# Autodesk Inventor assembly: Zebro_lotka
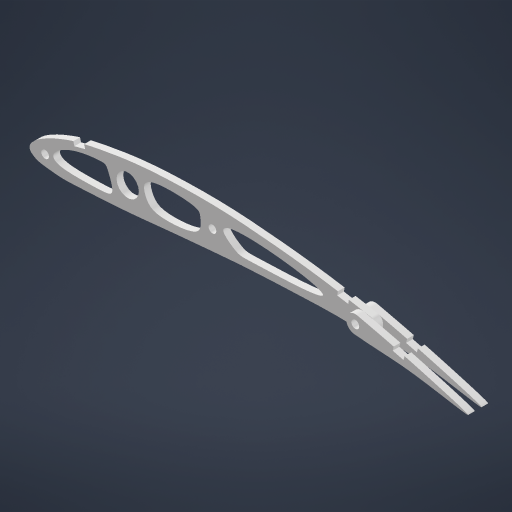
[picture p0: Inventor's stored thumbnail of the model, 512x512]
Saved by Autodesk Inventor 2023 (Build 270158000, 158)
## iProperties
Created: 2023-01-05
Part Number: Zebro_lotka
Document SubType Name: Assembly
Designer: szykr
Author: szykr
## Documents named in this file (3)
- D:\Folder Instalacyjny\GitHub Pliki\Solaris\new model\Zebro_lotka.iam
- D:\Folder Instalacyjny\GitHub Pliki\Solaris\new model\Żebro z lotką.ipt
- D:\Folder Instalacyjny\GitHub Pliki\Solaris\new model\Lotka.ipt
## Components (3 placed, 2 different names)
1. Żebro z lotką:1 — Rotational:1, Rotational:2
2. Lotka:1 — Rotational:2, Angle:1
3. Lotka:2 — Rotational:1, Angle:1
## Relationships (3: RevoluteJoint 2, Angle 1)
- Rotational:1 [RevoluteJoint]: Żebro z lotką:1 ↔ Lotka:2
- Rotational:2 [RevoluteJoint]: Żebro z lotką:1 ↔ Lotka:1
- Angle:1 (0 deg): Lotka:1 ↔ Lotka:2
